# Autodesk Inventor assembly: RPI_assembly
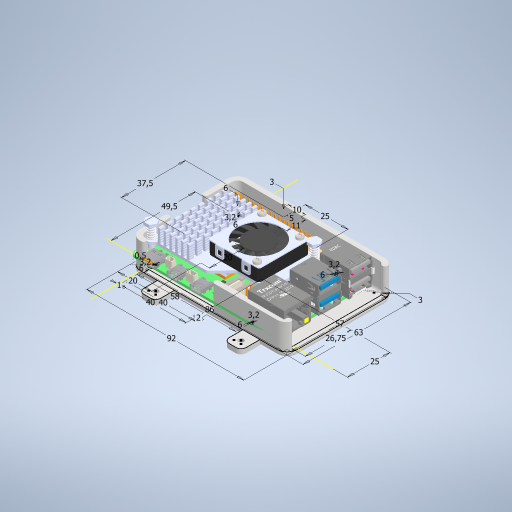
[picture p0: Inventor's stored thumbnail of the model, 512x512]
Saved by Autodesk Inventor 2024.3 (Build 283343000, 343)
## iProperties
Created: 2026-05-03
Part Number: RPI_assembly
Document SubType Name: Assembly
Designer: owozn
Author: owozn
## Documents named in this file (4)
- C:\Users\owozn\Documents\Nauka\Studia\mgr\Semestr_3\Magisterka\uMule\mechanics\subsets\attachments\raspberry_pi\RPI_assembly.iam
- C:\Users\owozn\Documents\Nauka\Studia\mgr\Semestr_3\Magisterka\uMule\mechanics\subsets\attachments\raspberry_pi\Raspberry_PI+fan\raspberry-pi-5-active-cooler-1.snapshot.1\Heatsink+fan RPi-5\Heatsink+fan RPi-5.iam
- C:\Users\owozn\Documents\Nauka\Studia\mgr\Semestr_3\Magisterka\uMule\mechanics\subsets\attachments\raspberry_pi\Raspberry_PI+fan\RASPBERRY_PI_5_1\RASPBERRY_PI_5_1.iam
- C:\Users\owozn\Documents\Nauka\Studia\mgr\Semestr_3\Magisterka\uMule\mechanics\subsets\attachments\raspberry_pi\RPi_case_bottom.ipt
## Components (3 placed, 3 different names)
1. Heatsink+fan RPi-5:1 [sub-assembly] — Mate:1, Mate:2, Mate:3
2. RASPBERRY_PI_5_1:1 [sub-assembly] — Mate:1, Mate:2, Mate:3, Flush:1, Flush:2, Mate:4
3. RPi_case_bottom:1 — Flush:1, Flush:2, Mate:4
## Relationships (6: Mate 4, Flush 2)
- Mate:1: Heatsink+fan RPi-5:1 ↔ RASPBERRY_PI_5_1:1
- Mate:2: Heatsink+fan RPi-5:1 ↔ RASPBERRY_PI_5_1:1
- Mate:3: Heatsink+fan RPi-5:1 ↔ RASPBERRY_PI_5_1:1
- Flush:1: RASPBERRY_PI_5_1:1 ↔ RPi_case_bottom:1
- Flush:2: RASPBERRY_PI_5_1:1 ↔ RPi_case_bottom:1
- Mate:4 (3 mm): RASPBERRY_PI_5_1:1 ↔ RPi_case_bottom:1
